# Autodesk Inventor assembly: wh_ass_3
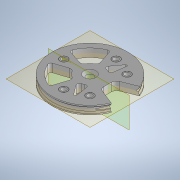
[picture p0: Inventor's stored thumbnail of the model, 180x180]
Saved by Autodesk Inventor 2020 (Build 240168000, 168)
## iProperties
Created: 2021-02-18
Part Number: wh_ass_3
Document SubType Name: Assembly
Designer: Shuang Peng
Author: Shuang Peng
## Documents named in this file (3)
- D:\projects-3\biped_tiny\hardware\wh_ass_3.iam
- D:\projects-3\biped_tiny\hardware\screw_holder_2_3.ipt
- D:\projects-3\biped_tiny\hardware\tendon_wh_3.ipt
## Components (6 placed, 2 different names)
1. screw_holder_2_3:1 — Insert:4
2. screw_holder_2_3:2 — Insert:3
3. screw_holder_2_3:3 — Insert:5
4. screw_holder_2_3:4 — Insert:1
5. screw_holder_2_3:5 — Insert:2
6. tendon_wh_3:1 — Insert:1, Insert:2, Insert:3, Insert:4, Insert:5
## Relationships (5: Insert 5)
- Insert:1: screw_holder_2_3:4 ↔ tendon_wh_3:1
- Insert:2: screw_holder_2_3:5 ↔ tendon_wh_3:1
- Insert:3: screw_holder_2_3:2 ↔ tendon_wh_3:1
- Insert:4: screw_holder_2_3:1 ↔ tendon_wh_3:1
- Insert:5: screw_holder_2_3:3 ↔ tendon_wh_3:1
